# Autodesk Inventor assembly: Ensamble_Carcasa4.0
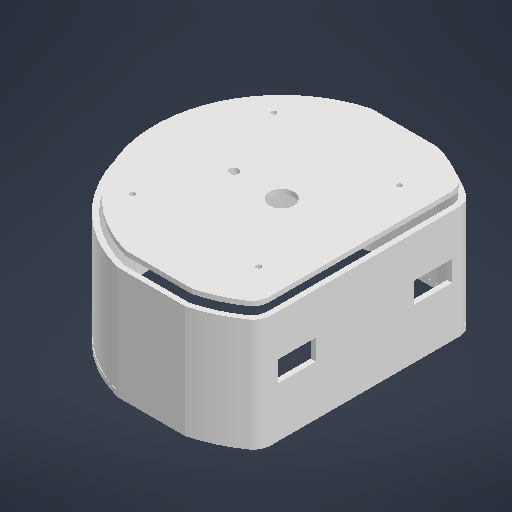
[picture p0: Inventor's stored thumbnail of the model, 512x512]
Saved by Autodesk Inventor 2026.2 (Build 302298000, 298)
## iProperties
Created: 2025-10-09
Part Number: Ensamble_Carcasa4.0
Document SubType Name: Assembly
Designer: brene
Author: brene
## Documents named in this file (3)
- C:\Users\06aar\Documents\Atta-Bot-STEM-Fork-aavalerin\Chasis\Diseño V3.0\Ensamble_Carcasa4.0.iam
- C:\Users\06aar\Documents\Atta-Bot-STEM-Fork-aavalerin\Chasis\Diseño V3.0\carcasa4.0.ipt
- C:\Users\06aar\Documents\Atta-Bot-STEM-Fork-aavalerin\Chasis\Diseño V3.0\tapa_carcasa_4.0.ipt
## Components (2 placed, 2 different names)
1. carcasa4.0:1 — Mate:1
2. tapa_carcasa_4.0:1 — Mate:1
## Relationships (1: Mate 1)
- Mate:1: carcasa4.0:1 ↔ tapa_carcasa_4.0:1
